# Autodesk Inventor assembly: iLogic_For_Dummies_Completed
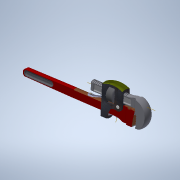
[picture p0: Inventor's stored thumbnail of the model, 180x180]
Saved by Autodesk Inventor 2020 (Build 240168000, 168)
## iProperties
Category: DATASETS
Manager: MANNY MANAGER
Company: ACME
RuleStatus: InUse
Created: 2009-12-11
Part Number: iLogic_For_Dummies_Completed
Document SubType Name: Assembly
Designer: JOE DESIGNER
Project: IV2010 TO 2011 UPDATE
Description: STILLSON WRENCH
Stock Number: F1496
Mass: 1878.1 g
Surface Area: 745.712 cm^2
Volume: 243.162 cm^3
Density: 7.72364 g/cm^3
Checked By: CHUCK CHECKER
Engr Approved By: ED ENGINEER
Mfg Approved By: DUNN RITE
Engineer: ERNIE ENGINEER
Author: Joe Designer
Revision Number: 0
Title: STILLSON WRENCH
Subject: Simplification for Simulation
Comments: To use for Exercise: Rules Using Spreadsheets, Forms, and Triggers
## Documents named in this file (9)
- C:\Dev\DaWrenchConfig\DaWrenchConfig\DebugPluginLocally\inputFiles\Wrench.iam
- C:\Dev\DaWrenchConfig\DaWrenchConfig\DebugPluginLocally\inputFiles\DS51F1496-02_Forms.ipt
- C:\Dev\DaWrenchConfig\DaWrenchConfig\DebugPluginLocally\inputFiles\DS51F1496-03_Forms.ipt
- C:\Dev\DaWrenchConfig\DaWrenchConfig\DebugPluginLocally\inputFiles\DS51F1496-04_Forms.ipt
- C:\Dev\DaWrenchConfig\DaWrenchConfig\DebugPluginLocally\inputFiles\DS51F1496-05_Forms.ipt
- C:\Dev\DaWrenchConfig\DaWrenchConfig\DebugPluginLocally\inputFiles\DS51F1496-06_Forms.ipt
- C:\Dev\DaWrenchConfig\DaWrenchConfig\DebugPluginLocally\inputFiles\DS51F1496-08_Forms.ipt
- C:\Dev\DaWrenchConfig\DaWrenchConfig\DebugPluginLocally\inputFiles\DS51F1496-07_Forms.ipt
- C:\Dev\DaWrenchConfig\DaWrenchConfig\DebugPluginLocally\inputFiles\Wrench_Bar_Complete.ipt
## Components (9 placed, 8 different names)
1. Wrench_Bar_Complete:1 — Mate:7, Mate:17, Flush:9, Mate:1, Flush:12, Mate:21, Mate:22, Flush:13, Mate:23, Mate:3, Angle:2, Mate:2, Flush:14, Angle:3
2. DS51F1496-02_Forms:1 — Mate:20, Flush:11, Rotation/Translation:1
3. DS51F1496-03_Forms:1 — Mate:19, Flush:11
4. DS51F1496-04_Forms:1 — Mate:19, Mate:20, Flush:12, Rotation/Translation:1, Mate:23
5. DS51F1496-05_Forms:1 — Mate:7, Flush:13
6. DS51F1496-06_Forms:1 — Mate:17, Flush:9, Angle:2
7. DS51F1496-07_Forms:1 — Mate:21, Mate:2
8. DS51F1496-07_Forms:2 — Mate:22, Mate:3
9. DS51F1496-08_Forms:1 — Mate:1, Flush:14, Angle:3
## Relationships (19: Mate 10, Flush 5, Angle 2, RelateRotateTranslate 1, Composite 1)
- Mate:17: Wrench_Bar_Complete:1 ↔ DS51F1496-06_Forms:1
- Flush:9: Wrench_Bar_Complete:1 ↔ DS51F1496-06_Forms:1
- Mate:1: Wrench_Bar_Complete:1 ↔ DS51F1496-08_Forms:1
- Mate:19: DS51F1496-03_Forms:1 ↔ DS51F1496-04_Forms:1
- Flush:11: DS51F1496-02_Forms:1 ↔ DS51F1496-03_Forms:1
- Flush:12: Wrench_Bar_Complete:1 ↔ DS51F1496-04_Forms:1
- Rotation/Translation:1 [RelateRotateTranslate] (127 mm): DS51F1496-02_Forms:1 ↔ DS51F1496-04_Forms:1
- Mate:21: Wrench_Bar_Complete:1 ↔ DS51F1496-07_Forms:1
- Mate:2 (0.7 mm): Wrench_Bar_Complete:1 ↔ DS51F1496-07_Forms:1
- Mate:22: Wrench_Bar_Complete:1 ↔ DS51F1496-07_Forms:2
- Mate:3 (0.7 mm): Wrench_Bar_Complete:1 ↔ DS51F1496-07_Forms:2
- Flush:13: Wrench_Bar_Complete:1 ↔ DS51F1496-05_Forms:1
- Mate:23 (10 mm): Wrench_Bar_Complete:1 ↔ DS51F1496-04_Forms:1
- Angle:2 (193 deg): Wrench_Bar_Complete:1 ↔ DS51F1496-06_Forms:1
- Flush:14: Wrench_Bar_Complete:1 ↔ DS51F1496-08_Forms:1
- Angle:3 (180.5 deg): Wrench_Bar_Complete:1 ↔ DS51F1496-08_Forms:1
- Mate:7: Wrench_Bar_Complete:1 ↔ DS51F1496-05_Forms:1
- [Composite]: Wrench_Bar_Complete:1 ↔ DS51F1496-03_Forms:1
- Mate:20: DS51F1496-02_Forms:1 ↔ DS51F1496-04_Forms:1
